# Autodesk Inventor assembly: belt_linear
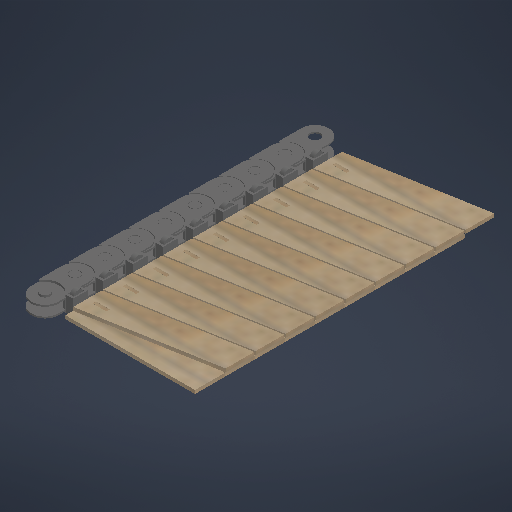
[picture p0: Inventor's stored thumbnail of the model, 512x512]
Saved by Autodesk Inventor 2026.1 (Build 301233020, 233B)
## iProperties
Created: 2025-09-27
Part Number: belt_linear
Document SubType Name: Assembly
Designer: hibik
Author: hibik
## Documents named in this file (3)
- C:\Users\hibik\Documents\Robomech\conveyer\belt\belt_linear.iam
- C:\Users\hibik\Documents\Robomech\conveyer\belt\belt.ipt
- C:\Users\hibik\Documents\Robomech\conveyer\belt\dish.iam
## Components (18 placed, 2 different names)
1. belt:1 — 挿入:1, 角度:9, メイト:1, メイト:2, メイト:3
2. belt:2 — 挿入:1, 挿入:2, 角度:9, 角度:10
3. belt:3 — 挿入:2, 挿入:3, 角度:10, 角度:11
4. belt:4 — 挿入:3, 挿入:16, 角度:11, 角度:12
5. belt:5 — 挿入:16, 角度:12, 角度:13
6. belt:6 — 角度:13, 角度:14
7. belt:7 — 角度:14, 角度:15
8. belt:8 — 角度:15, 挿入:18, 角度:17
9. belt:9 — 挿入:18, 角度:17
10. dish:1 [sub-assembly] — メイト:1, メイト:2, メイト:3, メイト:4, メイト:19, フラッシュ:8
11. dish:2 [sub-assembly] — メイト:4, メイト:5, フラッシュ:1, メイト:6, メイト:19, フラッシュ:8
12. dish:3 [sub-assembly] — メイト:5, フラッシュ:1, メイト:6, メイト:9, フラッシュ:3, メイト:10
13. dish:4 [sub-assembly] — メイト:9, フラッシュ:3, メイト:10
14. dish:5 [sub-assembly] — メイト:17, フラッシュ:7, メイト:18
15. dish:6 [sub-assembly] — メイト:17, フラッシュ:7, メイト:18
16. dish:7 [sub-assembly]
17. dish:8 [sub-assembly]
18. dish:9 [sub-assembly]
## Relationships (43: Mate 19, Insert 8, Angle 8, Flush 8)
- 挿入:1 [Insert] (0.6 mm): belt:1 ↔ belt:2
- 挿入:2 [Insert] (0.6 mm): belt:2 ↔ belt:3
- 挿入:3 [Insert] (0.6 mm): belt:3 ↔ belt:4
- [Insert] (0.6 mm): belt:5 ↔ belt:6
- [Insert] (0.6 mm): belt:6 ↔ belt:7
- [Insert] (0.6 mm): belt:7 ↔ belt:8
- 挿入:16 [Insert] (0.6 mm): belt:4 ↔ belt:5
- 角度:9 [Angle] (0 deg): belt:1 ↔ belt:2
- 角度:10 [Angle] (0 deg): belt:2 ↔ belt:3
- 角度:11 [Angle] (0 deg): belt:3 ↔ belt:4
- 角度:12 [Angle] (0 deg): belt:4 ↔ belt:5
- 角度:13 [Angle] (0 deg): belt:5 ↔ belt:6
- 角度:14 [Angle] (0 deg): belt:6 ↔ belt:7
- 角度:15 [Angle] (0 deg): belt:7 ↔ belt:8
- 挿入:18 [Insert] (0.6 mm): belt:8 ↔ belt:9
- 角度:17 [Angle] (0 deg): belt:8 ↔ belt:9
- メイト:1 [Mate]: belt:1 ↔ dish:1
- メイト:2 [Mate]: belt:1 ↔ dish:1
- メイト:3 [Mate]: belt:1 ↔ dish:1
- メイト:4 [Mate]: dish:1 ↔ dish:2
- メイト:5 [Mate]: dish:2 ↔ dish:3
- フラッシュ:1 [Flush]: dish:2 ↔ dish:3
- メイト:6 [Mate]: dish:2 ↔ dish:3
- [Mate]: dish:4 ↔ dish:5
- [Flush]: dish:4 ↔ dish:5
- [Mate]: dish:4 ↔ dish:5
- メイト:9 [Mate]: dish:3 ↔ dish:4
- フラッシュ:3 [Flush]: dish:3 ↔ dish:4
- メイト:10 [Mate]: dish:3 ↔ dish:4
- [Mate]: dish:6 ↔ dish:7
- [Flush]: dish:6 ↔ dish:7
- [Mate]: dish:6 ↔ dish:7
- [Mate]: dish:8 ↔ dish:9
- [Flush]: dish:8 ↔ dish:9
- [Mate]: dish:8 ↔ dish:9
- [Mate]: dish:7 ↔ dish:8
- [Flush]: dish:7 ↔ dish:8
- [Mate]: dish:7 ↔ dish:8
- メイト:17 [Mate]: dish:5 ↔ dish:6
- フラッシュ:7 [Flush]: dish:5 ↔ dish:6
- メイト:18 [Mate]: dish:5 ↔ dish:6
- メイト:19 [Mate]: dish:1 ↔ dish:2
- フラッシュ:8 [Flush]: dish:1 ↔ dish:2
## Named parameters: d12_d0 = 0.6 mm, d13_d1 = 0.6 mm, d14_d2 = 0.6 mm, d42_d39 = 0 mm, d43_d40 = 0 mm, d44_d41 = 0 mm, d48_d39 = 0 mm, d49_d40 = 0 mm, d50_d41 = 0 mm, d51_d42_d39 = 0 mm, d52_d43_d40 = 0 mm, d53_d44_d41 = 0 mm, d54_d45 = 0 mm, d55_d46 = 0 mm, d56_d47 = 0 mm
